# Autodesk Inventor assembly: MeasurementChamber Frame Assembly - Bade v4
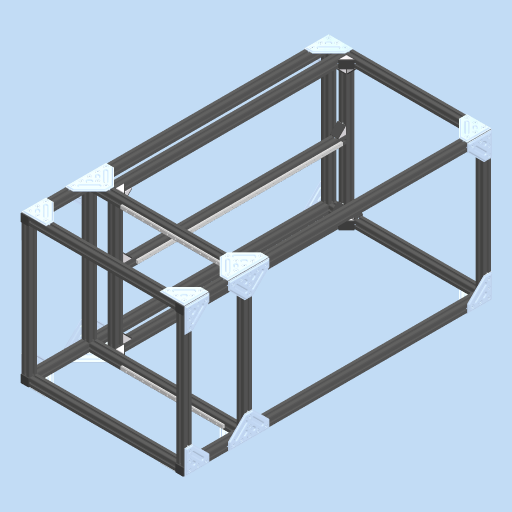
[picture p0: Inventor's stored thumbnail of the model, 512x512]
Saved by Autodesk Inventor 2023.2 (Build 272271000, 271)
## iProperties
Created: 2023-11-22
Part Number: MeasurementChamber Frame Assembly - Bade v4
Document SubType Name: Assembly
Designer: Nils Bade
Author: Nils Bade
## Documents named in this file (16)
- C:\Users\nilsb\Documents\Inventor\Projektarbeit-Bade\ITEM\ITEM Frame Assembly - Bade v1.iam
- ITEM Frame Assembly - Bade v1.iam
- C:\Users\nilsb\Documents\Inventor\Projektarbeit-Bade\ITEM\4040 Profile\ITEM T-SLOT 4040 715mm.ipt
- C:\Users\nilsb\Documents\Inventor\Projektarbeit-Bade\ITEM\4040 Profile\ITEM T-SLOT 4040 1500mm.ipt
- C:\Users\nilsb\Documents\Inventor\Projektarbeit-Bade\ITEM\4040 Profile\ITEM T-SLOT 4040 640mm.ipt
- C:\Users\nilsb\Documents\Inventor\Projektarbeit-Bade\ITEM\4040 Profile\ITEM T-SLOT 4040 1127mm.ipt
- C:\Users\nilsb\Documents\Inventor\Projektarbeit-Bade\ITEM\4040 Profile\ITEM T-SLOT 4040 1087mm.ipt
- C:\Users\nilsb\Documents\Inventor\Projektarbeit-Bade\ITEM\ITEM_41115_Winkelsatz_90er.iam
- C:\Users\nilsb\Documents\Inventor\Projektarbeit-Bade\ITEM\ITEM_0070805_T-Knotenblechsatz 8 40 200x120.ipt
- ITEM_0070805_T-Knotenblechsatz 8 40 200x120.ipt
- C:\Users\nilsb\Documents\Inventor\Projektarbeit-Bade\ITEM\ITEM_0070802_90erKnotenblechsatz 8 40 120x120.ipt
- C:\Users\nilsb\Documents\Inventor\Projektarbeit-Bade\ITEM\ITEM_0070805_T-Knotenblechsatz 8 40 200x120_MIR.ipt
- C:\Users\nilsb\Documents\Inventor\Projektarbeit-Bade\ITEM\ITEM_0070802_90erKnotenblechsatz 8 40 120x120_MIR.ipt
- C:\Users\nilsb\Documents\Inventor\Projektarbeit-Bade\RatRig_modified\MGN15 Linear Rail 1000mm - 4040 Assembly.iam
- C:\Users\nilsb\Documents\Inventor\Projektarbeit-Bade\RatRig_modified\MGN15 Linear Rail 500mm - 4040 Assembly.iam
- C:\Users\nilsb\Documents\Inventor\Projektarbeit-Bade\ITEM\ITEM_Abdeckkappe-40x40-schw_2601.ipt
## Components (66 placed, 13 different names)
1. ITEM T-SLOT 4040 1500mm:1 — Passend:162, Passend:163, Fluchtend:165, Passend:165, Fluchtend:19, Fluchtend:20, Passend:174, Fluchtend:166, Fluchtend:195, Passend:192, Passend:225, Passend:226, Passend:227, Passend:228, Passend:232, Passend:233, Passend:234, Passend:246, Passend:247, Passend:249, Passend:250, Passend:265, Fluchtend:267, Fluchtend:268
2. ITEM T-SLOT 4040 1500mm:2 — Passend:166, Passend:167, Passend:168, Fluchtend:167, Fluchtend:171, Passend:183, Passend:185, Fluchtend:188, Fluchtend:228, Passend:223, Passend:229, Passend:230, Fluchtend:233, Passend:238, Fluchtend:235, Passend:240, Passend:242, Passend:257, Fluchtend:259, Passend:262, Fluchtend:261, Fluchtend:262, Passend:263
3. ITEM T-SLOT 4040 1500mm:3 — Fluchtend:168, Passend:176, Passend:178, Passend:181, Fluchtend:193, Passend:190, Fluchtend:196, Fluchtend:200, Passend:266, Fluchtend:265, Fluchtend:266
4. ITEM T-SLOT 4040 1500mm:4 — Passend:177, Fluchtend:169, Passend:179, Fluchtend:170, Passend:184, Fluchtend:186, Fluchtend:187, Fluchtend:189, Passend:186, Fluchtend:197, Fluchtend:198, Passend:191, Fluchtend:201, Passend:193, Symmetrie:1, Fluchtend:238, Passend:256, Fluchtend:263, Fluchtend:264, Passend:264
5. ITEM T-SLOT 4040 715mm:1 — Passend:165, Fluchtend:19, Fluchtend:20, Passend:168, Passend:172, Passend:173, Fluchtend:194, Passend:188, Fluchtend:207, Fluchtend:210, Fluchtend:215, Passend:200, Passend:201, Fluchtend:236, Fluchtend:237
6. ITEM T-SLOT 4040 715mm:2 — Passend:180, Fluchtend:170, Passend:181, Passend:187, Fluchtend:206, Fluchtend:211, Passend:209, Fluchtend:219, Passend:212
7. ITEM T-SLOT 4040 715mm:3 — Fluchtend:171, Passend:182, Passend:183, Passend:231, Passend:236, Passend:237
8. ITEM T-SLOT 4040 715mm:4 — Passend:184, Fluchtend:186, Fluchtend:187
9. ITEM T-SLOT 4040 715mm:5 — Passend:185, Fluchtend:188, Fluchtend:190, Passend:195, Passend:216, Fluchtend:227, Passend:224, Fluchtend:229
10. ITEM T-SLOT 4040 715mm:6 — Fluchtend:189, Passend:186, Fluchtend:190, Passend:189, Fluchtend:199, Fluchtend:202, Passend:222
11. ITEM T-SLOT 4040 640mm:1 — Passend:171, Passend:172, Fluchtend:167, Passend:175, Fluchtend:169, Passend:179, Fluchtend:205, Fluchtend:212, Fluchtend:213, Passend:241, Passend:243
12. ITEM T-SLOT 4040 640mm:2 — Passend:170, Passend:173, Passend:175, Fluchtend:191, Fluchtend:192, Fluchtend:209, Fluchtend:214, Passend:202, Fluchtend:216, Passend:203, Fluchtend:217, Passend:205, Fluchtend:218, Passend:207, Passend:208, Fluchtend:220, Fluchtend:221
13. ITEM T-SLOT 4040 640mm:3 — Passend:169, Passend:174, Fluchtend:166, Passend:178, Passend:248
14. ITEM T-SLOT 4040 640mm:4 — Passend:194, Passend:195, Fluchtend:203, Fluchtend:208, Passend:215, Passend:217, Passend:219, Fluchtend:225
15. ITEM T-SLOT 4040 640mm:5 — Fluchtend:199, Fluchtend:200, Passend:192
16. ITEM T-SLOT 4040 640mm:6 — Fluchtend:201, Passend:193, Fluchtend:202, Fluchtend:231
17. ITEM T-SLOT 4040 640mm:7 — Fluchtend:197, Fluchtend:198, Passend:191, Fluchtend:234, Passend:239
18. ITEM T-SLOT 4040 640mm:8 — Fluchtend:195, Passend:190, Fluchtend:196, Fluchtend:232, Passend:235
19. ITEM T-SLOT 4040 1127mm:2 — Fluchtend:192, Fluchtend:193, Passend:187, Passend:189, Passend:210, Passend:211, Passend:220, Passend:221, Fluchtend:226
20. ITEM T-SLOT 4040 1127mm:1 — Fluchtend:191, Fluchtend:194, Passend:188, Passend:194, Fluchtend:203, Passend:199, Passend:204, Passend:213, Passend:214, Fluchtend:222, Fluchtend:223
21. ITEM T-SLOT 4040 1087mm:1 — Passend:206, Passend:218, Fluchtend:224, Passend:254, Passend:255
22. ITEM_Abdeckkappe-40x40-schw_2601:1 — Fluchtend:261, Fluchtend:262, Passend:263
23. ITEM_Abdeckkappe-40x40-schw_2601:2 — Fluchtend:263, Fluchtend:264, Passend:264
24. ITEM_Abdeckkappe-40x40-schw_2601:3 — Passend:265, Fluchtend:267, Fluchtend:268
25. ITEM_Abdeckkappe-40x40-schw_2601:4 — Passend:266, Fluchtend:265, Fluchtend:266
26. ITEM_41115_Winkelsatz_90er:1 [sub-assembly] — Fluchtend:215, Passend:199, Passend:200
27. ITEM_41115_Winkelsatz_90er:2 [sub-assembly] — Passend:203, Fluchtend:217, Passend:204
28. ITEM_41115_Winkelsatz_90er:3 [sub-assembly] — Passend:201, Passend:202, Fluchtend:216
29. ITEM_41115_Winkelsatz_90er:4 [sub-assembly] — Passend:205, Passend:206, Fluchtend:218
30. ITEM_41115_Winkelsatz_90er:5 [sub-assembly] — Passend:207, Fluchtend:220, Passend:211
31. ITEM_41115_Winkelsatz_90er:6 [sub-assembly] — Passend:208, Fluchtend:221, Passend:212
32. ITEM_41115_Winkelsatz_90er:7 [sub-assembly] — Passend:209, Passend:210, Fluchtend:219
33. ITEM_41115_Winkelsatz_90er:8 [sub-assembly] — Passend:213, Fluchtend:223, Passend:216
34. ITEM_41115_Winkelsatz_90er:9 [sub-assembly] — Passend:214, Passend:215, Fluchtend:222
35. ITEM_41115_Winkelsatz_90er:10 [sub-assembly] — Passend:217, Passend:218, Fluchtend:224
36. ITEM_41115_Winkelsatz_90er:11 [sub-assembly] — Passend:219, Passend:220, Fluchtend:225
37. ITEM_41115_Winkelsatz_90er:12 [sub-assembly] — Passend:221, Passend:222, Fluchtend:226
38. ITEM_0070805_T-Knotenblechsatz 8 40 200x120:1 — Passend:224, Passend:225, Passend:226
39. ITEM_0070805_T-Knotenblechsatz 8 40 200x120:2 — Fluchtend:227, Fluchtend:228, Passend:223
40. ITEM_0070805_T-Knotenblechsatz 8 40 200x120:3 — Fluchtend:229, Passend:227, Passend:228
41. ITEM_0070805_T-Knotenblechsatz 8 40 200x120:4 — Passend:229, Fluchtend:231, Passend:230
42. ITEM_0070802_90erKnotenblechsatz 8 40 120x120:1 — Passend:231, Passend:232, Passend:233
43. ITEM_0070802_90erKnotenblechsatz 8 40 120x120:2 — Passend:234, Fluchtend:232, Passend:235
44. ITEM_0070802_90erKnotenblechsatz 8 40 120x120:3 — Fluchtend:234, Passend:238, Passend:239
45. ITEM_0070802_90erKnotenblechsatz 8 40 120x120:4 — Passend:236, Fluchtend:233, Passend:237
46. ITEM_0070802_90erKnotenblechsatz 8 40 120x120:5 — Fluchtend:235, Fluchtend:236, Passend:240
47. ITEM_0070802_90erKnotenblechsatz 8 40 120x120:6 — Passend:246, Fluchtend:237, Passend:250
48. ITEM_0070802_90erKnotenblechsatz 8 40 120x120:7 — Passend:241, Passend:242, Passend:243
49. ITEM_0070802_90erKnotenblechsatz 8 40 120x120:8 — Passend:247, Passend:248, Passend:249
50. ITEM_0070805_T-Knotenblechsatz 8 40 200x120_MIR:1
51. ITEM_0070805_T-Knotenblechsatz 8 40 200x120_MIR:2
52. ITEM_0070805_T-Knotenblechsatz 8 40 200x120_MIR:3
53. ITEM_0070805_T-Knotenblechsatz 8 40 200x120_MIR:4
54. ITEM_0070802_90erKnotenblechsatz 8 40 120x120_MIR:1
55. ITEM_0070802_90erKnotenblechsatz 8 40 120x120_MIR:2
56. ITEM_0070802_90erKnotenblechsatz 8 40 120x120_MIR:3
57. ITEM_0070802_90erKnotenblechsatz 8 40 120x120_MIR:4
58. ITEM_0070802_90erKnotenblechsatz 8 40 120x120_MIR:5
59. ITEM_0070802_90erKnotenblechsatz 8 40 120x120_MIR:6
60. ITEM_0070802_90erKnotenblechsatz 8 40 120x120_MIR:7
61. ITEM_0070802_90erKnotenblechsatz 8 40 120x120_MIR:8
62. MGN15 Linear Rail 1000mm - 4040 Assembly:1 [sub-assembly] — Passend:253, Fluchtend:238, Passend:256
63. MGN15 Linear Rail 1000mm - 4040 Assembly:2 [sub-assembly] — Passend:252, Passend:257, Fluchtend:259
64. MGN15 Linear Rail 1000mm - 4040 Assembly:3 [sub-assembly] — Passend:251, Passend:254, Passend:255
65. MGN15 Linear Rail 500mm - 4040 Assembly:1 [sub-assembly] — Passend:262
66. MGN15 Linear Rail 500mm - 4040 Assembly:2 [sub-assembly]
## Relationships (180: Mate 105, Flush 74, Symmetry 1)
- Fluchtend:17 [Flush] (1057 mm)
- Passend:156 [Mate]
- Passend:157 [Mate]
- Passend:158 [Mate]
- Passend:159 [Mate]
- Passend:160 [Mate]
- Passend:161 [Mate]
- Passend:162 [Mate]: ITEM T-SLOT 4040 1500mm:1
- Passend:163 [Mate]: ITEM T-SLOT 4040 1500mm:1
- Fluchtend:165 [Flush]: ITEM T-SLOT 4040 1500mm:1
- Passend:165 [Mate]: ITEM T-SLOT 4040 1500mm:1 ↔ ITEM T-SLOT 4040 715mm:1
- Fluchtend:19 [Flush]: ITEM T-SLOT 4040 1500mm:1 ↔ ITEM T-SLOT 4040 715mm:1
- Fluchtend:20 [Flush]: ITEM T-SLOT 4040 1500mm:1 ↔ ITEM T-SLOT 4040 715mm:1
- Passend:166 [Mate]: ITEM T-SLOT 4040 1500mm:2
- Passend:167 [Mate]: ITEM T-SLOT 4040 1500mm:2
- Passend:168 [Mate]: ITEM T-SLOT 4040 1500mm:2 ↔ ITEM T-SLOT 4040 715mm:1
- Passend:169 [Mate]: ITEM T-SLOT 4040 640mm:3
- Passend:170 [Mate]: ITEM T-SLOT 4040 640mm:2
- Passend:171 [Mate]: ITEM T-SLOT 4040 640mm:1
- Passend:172 [Mate]: ITEM T-SLOT 4040 715mm:1 ↔ ITEM T-SLOT 4040 640mm:1
- Passend:173 [Mate]: ITEM T-SLOT 4040 715mm:1 ↔ ITEM T-SLOT 4040 640mm:2
- Passend:174 [Mate]: ITEM T-SLOT 4040 1500mm:1 ↔ ITEM T-SLOT 4040 640mm:3
- Fluchtend:166 [Flush]: ITEM T-SLOT 4040 1500mm:1 ↔ ITEM T-SLOT 4040 640mm:3
- Fluchtend:167 [Flush]: ITEM T-SLOT 4040 1500mm:2 ↔ ITEM T-SLOT 4040 640mm:1
- Passend:175 [Mate] (628 mm): ITEM T-SLOT 4040 640mm:1 ↔ ITEM T-SLOT 4040 640mm:2
- Fluchtend:168 [Flush]: ITEM T-SLOT 4040 1500mm:3
- Passend:176 [Mate]: ITEM T-SLOT 4040 1500mm:3
- Passend:177 [Mate]: ITEM T-SLOT 4040 1500mm:4
- Passend:178 [Mate]: ITEM T-SLOT 4040 1500mm:3 ↔ ITEM T-SLOT 4040 640mm:3
- Fluchtend:169 [Flush]: ITEM T-SLOT 4040 1500mm:4 ↔ ITEM T-SLOT 4040 640mm:1
- Passend:179 [Mate]: ITEM T-SLOT 4040 1500mm:4 ↔ ITEM T-SLOT 4040 640mm:1
- Passend:180 [Mate]: ITEM T-SLOT 4040 715mm:2
- Fluchtend:170 [Flush]: ITEM T-SLOT 4040 1500mm:4 ↔ ITEM T-SLOT 4040 715mm:2
- Passend:181 [Mate]: ITEM T-SLOT 4040 1500mm:3 ↔ ITEM T-SLOT 4040 715mm:2
- Fluchtend:171 [Flush]: ITEM T-SLOT 4040 1500mm:2 ↔ ITEM T-SLOT 4040 715mm:3
- Passend:182 [Mate]: ITEM T-SLOT 4040 715mm:3
- Passend:183 [Mate]: ITEM T-SLOT 4040 1500mm:2 ↔ ITEM T-SLOT 4040 715mm:3
- Passend:184 [Mate]: ITEM T-SLOT 4040 1500mm:4 ↔ ITEM T-SLOT 4040 715mm:4
- Fluchtend:186 [Flush]: ITEM T-SLOT 4040 1500mm:4 ↔ ITEM T-SLOT 4040 715mm:4
- Fluchtend:187 [Flush]: ITEM T-SLOT 4040 1500mm:4 ↔ ITEM T-SLOT 4040 715mm:4
- Passend:185 [Mate]: ITEM T-SLOT 4040 1500mm:2 ↔ ITEM T-SLOT 4040 715mm:5
- Fluchtend:188 [Flush]: ITEM T-SLOT 4040 1500mm:2 ↔ ITEM T-SLOT 4040 715mm:5
- Fluchtend:189 [Flush]: ITEM T-SLOT 4040 1500mm:4 ↔ ITEM T-SLOT 4040 715mm:6
- Passend:186 [Mate]: ITEM T-SLOT 4040 1500mm:4 ↔ ITEM T-SLOT 4040 715mm:6
- Fluchtend:190 [Flush]: ITEM T-SLOT 4040 715mm:5 ↔ ITEM T-SLOT 4040 715mm:6
- Fluchtend:191 [Flush]: ITEM T-SLOT 4040 640mm:2 ↔ ITEM T-SLOT 4040 1127mm:1
- Fluchtend:192 [Flush]: ITEM T-SLOT 4040 640mm:2 ↔ ITEM T-SLOT 4040 1127mm:2
- Fluchtend:193 [Flush]: ITEM T-SLOT 4040 1500mm:3 ↔ ITEM T-SLOT 4040 1127mm:2
- Passend:187 [Mate]: ITEM T-SLOT 4040 715mm:2 ↔ ITEM T-SLOT 4040 1127mm:2
- Fluchtend:194 [Flush]: ITEM T-SLOT 4040 715mm:1 ↔ ITEM T-SLOT 4040 1127mm:1
- Passend:188 [Mate]: ITEM T-SLOT 4040 715mm:1 ↔ ITEM T-SLOT 4040 1127mm:1
- Passend:189 [Mate]: ITEM T-SLOT 4040 715mm:6 ↔ ITEM T-SLOT 4040 1127mm:2
- Fluchtend:195 [Flush]: ITEM T-SLOT 4040 1500mm:1 ↔ ITEM T-SLOT 4040 640mm:8
- Passend:190 [Mate]: ITEM T-SLOT 4040 1500mm:3 ↔ ITEM T-SLOT 4040 640mm:8
- Fluchtend:196 [Flush]: ITEM T-SLOT 4040 1500mm:3 ↔ ITEM T-SLOT 4040 640mm:8
- Fluchtend:197 [Flush]: ITEM T-SLOT 4040 1500mm:4 ↔ ITEM T-SLOT 4040 640mm:7
- Fluchtend:198 [Flush]: ITEM T-SLOT 4040 1500mm:4 ↔ ITEM T-SLOT 4040 640mm:7
- Passend:191 [Mate]: ITEM T-SLOT 4040 1500mm:4 ↔ ITEM T-SLOT 4040 640mm:7
- Fluchtend:199 [Flush]: ITEM T-SLOT 4040 715mm:6 ↔ ITEM T-SLOT 4040 640mm:5
- Fluchtend:200 [Flush]: ITEM T-SLOT 4040 1500mm:3 ↔ ITEM T-SLOT 4040 640mm:5
- Passend:192 [Mate]: ITEM T-SLOT 4040 1500mm:1 ↔ ITEM T-SLOT 4040 640mm:5
- Fluchtend:201 [Flush]: ITEM T-SLOT 4040 1500mm:4 ↔ ITEM T-SLOT 4040 640mm:6
- Passend:193 [Mate]: ITEM T-SLOT 4040 1500mm:4 ↔ ITEM T-SLOT 4040 640mm:6
- Fluchtend:202 [Flush]: ITEM T-SLOT 4040 715mm:6 ↔ ITEM T-SLOT 4040 640mm:6
- Passend:194 [Mate]: ITEM T-SLOT 4040 640mm:4 ↔ ITEM T-SLOT 4040 1127mm:1
- Passend:195 [Mate]: ITEM T-SLOT 4040 715mm:5 ↔ ITEM T-SLOT 4040 640mm:4
- Fluchtend:203 [Flush]: ITEM T-SLOT 4040 640mm:4 ↔ ITEM T-SLOT 4040 1127mm:1
- [Mate]: ITEM T-SLOT 4040 640mm:2 ↔ ITEM T-SLOT 4040 1087mm:1
- [Flush]: ITEM T-SLOT 4040 640mm:2 ↔ ITEM T-SLOT 4040 1087mm:1
- Symmetrie:1: ITEM T-SLOT 4040 1500mm:4
- [Mate]: ITEM T-SLOT 4040 1087mm:1
- Fluchtend:205 [Flush] (21.5 mm): ITEM T-SLOT 4040 640mm:1
- Fluchtend:206 [Flush] (21.5 mm): ITEM T-SLOT 4040 715mm:2
- Fluchtend:207 [Flush] (21.5 mm): ITEM T-SLOT 4040 715mm:1
- Fluchtend:208 [Flush] (35.5 mm): ITEM T-SLOT 4040 640mm:4
- Fluchtend:209 [Flush] (70 mm): ITEM T-SLOT 4040 640mm:2
- Fluchtend:210 [Flush] (51.86 mm): ITEM T-SLOT 4040 715mm:1
- Fluchtend:211 [Flush] (51.86 mm): ITEM T-SLOT 4040 715mm:2
- Fluchtend:212 [Flush] (25.242 mm): ITEM T-SLOT 4040 640mm:1
- Fluchtend:213 [Flush] (47 mm): ITEM T-SLOT 4040 640mm:1
- Fluchtend:214 [Flush] (27 mm): ITEM T-SLOT 4040 640mm:2
- Fluchtend:215 [Flush]: ITEM T-SLOT 4040 715mm:1 ↔ ITEM_41115_Winkelsatz_90er:1
- Passend:199 [Mate]: ITEM T-SLOT 4040 1127mm:1 ↔ ITEM_41115_Winkelsatz_90er:1
- Passend:200 [Mate]: ITEM T-SLOT 4040 715mm:1 ↔ ITEM_41115_Winkelsatz_90er:1
- Passend:201 [Mate]: ITEM T-SLOT 4040 715mm:1 ↔ ITEM_41115_Winkelsatz_90er:3
- Passend:202 [Mate]: ITEM T-SLOT 4040 640mm:2 ↔ ITEM_41115_Winkelsatz_90er:3
- Fluchtend:216 [Flush]: ITEM T-SLOT 4040 640mm:2 ↔ ITEM_41115_Winkelsatz_90er:3
- Passend:203 [Mate]: ITEM T-SLOT 4040 640mm:2 ↔ ITEM_41115_Winkelsatz_90er:2
- Fluchtend:217 [Flush]: ITEM T-SLOT 4040 640mm:2 ↔ ITEM_41115_Winkelsatz_90er:2
- Passend:204 [Mate]: ITEM T-SLOT 4040 1127mm:1 ↔ ITEM_41115_Winkelsatz_90er:2
- Passend:205 [Mate]: ITEM T-SLOT 4040 640mm:2 ↔ ITEM_41115_Winkelsatz_90er:4
- Passend:206 [Mate]: ITEM T-SLOT 4040 1087mm:1 ↔ ITEM_41115_Winkelsatz_90er:4
- Fluchtend:218 [Flush]: ITEM T-SLOT 4040 640mm:2 ↔ ITEM_41115_Winkelsatz_90er:4
- Passend:207 [Mate]: ITEM T-SLOT 4040 640mm:2 ↔ ITEM_41115_Winkelsatz_90er:5
- Passend:208 [Mate]: ITEM T-SLOT 4040 640mm:2 ↔ ITEM_41115_Winkelsatz_90er:6
- Passend:209 [Mate]: ITEM T-SLOT 4040 715mm:2 ↔ ITEM_41115_Winkelsatz_90er:7
- Passend:210 [Mate]: ITEM T-SLOT 4040 1127mm:2 ↔ ITEM_41115_Winkelsatz_90er:7
- Fluchtend:219 [Flush]: ITEM T-SLOT 4040 715mm:2 ↔ ITEM_41115_Winkelsatz_90er:7
- Fluchtend:220 [Flush]: ITEM T-SLOT 4040 640mm:2 ↔ ITEM_41115_Winkelsatz_90er:5
- Fluchtend:221 [Flush]: ITEM T-SLOT 4040 640mm:2 ↔ ITEM_41115_Winkelsatz_90er:6
- Passend:211 [Mate]: ITEM T-SLOT 4040 1127mm:2 ↔ ITEM_41115_Winkelsatz_90er:5
- Passend:212 [Mate]: ITEM T-SLOT 4040 715mm:2 ↔ ITEM_41115_Winkelsatz_90er:6
- Passend:213 [Mate]: ITEM T-SLOT 4040 1127mm:1 ↔ ITEM_41115_Winkelsatz_90er:8
- Passend:214 [Mate]: ITEM T-SLOT 4040 1127mm:1 ↔ ITEM_41115_Winkelsatz_90er:9
- Passend:215 [Mate]: ITEM T-SLOT 4040 640mm:4 ↔ ITEM_41115_Winkelsatz_90er:9
- Fluchtend:222 [Flush]: ITEM T-SLOT 4040 1127mm:1 ↔ ITEM_41115_Winkelsatz_90er:9
- Fluchtend:223 [Flush]: ITEM T-SLOT 4040 1127mm:1 ↔ ITEM_41115_Winkelsatz_90er:8
- Passend:216 [Mate]: ITEM T-SLOT 4040 715mm:5 ↔ ITEM_41115_Winkelsatz_90er:8
- Passend:217 [Mate]: ITEM T-SLOT 4040 640mm:4 ↔ ITEM_41115_Winkelsatz_90er:10
- Passend:218 [Mate]: ITEM T-SLOT 4040 1087mm:1 ↔ ITEM_41115_Winkelsatz_90er:10
- Fluchtend:224 [Flush]: ITEM T-SLOT 4040 1087mm:1 ↔ ITEM_41115_Winkelsatz_90er:10
- Passend:219 [Mate]: ITEM T-SLOT 4040 640mm:4 ↔ ITEM_41115_Winkelsatz_90er:11
- Passend:220 [Mate]: ITEM T-SLOT 4040 1127mm:2 ↔ ITEM_41115_Winkelsatz_90er:11
- Fluchtend:225 [Flush]: ITEM T-SLOT 4040 640mm:4 ↔ ITEM_41115_Winkelsatz_90er:11
- Passend:221 [Mate]: ITEM T-SLOT 4040 1127mm:2 ↔ ITEM_41115_Winkelsatz_90er:12
- Passend:222 [Mate]: ITEM T-SLOT 4040 715mm:6 ↔ ITEM_41115_Winkelsatz_90er:12
- Fluchtend:226 [Flush]: ITEM T-SLOT 4040 1127mm:2 ↔ ITEM_41115_Winkelsatz_90er:12
- Fluchtend:227 [Flush]: ITEM T-SLOT 4040 715mm:5 ↔ ITEM_0070805_T-Knotenblechsatz 8 40 200x120:2
- Fluchtend:228 [Flush]: ITEM T-SLOT 4040 1500mm:2 ↔ ITEM_0070805_T-Knotenblechsatz 8 40 200x120:2
- Passend:223 [Mate]: ITEM T-SLOT 4040 1500mm:2 ↔ ITEM_0070805_T-Knotenblechsatz 8 40 200x120:2
- Passend:224 [Mate]: ITEM T-SLOT 4040 715mm:5 ↔ ITEM_0070805_T-Knotenblechsatz 8 40 200x120:1
- Passend:225 [Mate]: ITEM T-SLOT 4040 1500mm:1 ↔ ITEM_0070805_T-Knotenblechsatz 8 40 200x120:1
- Passend:226 [Mate]: ITEM T-SLOT 4040 1500mm:1 ↔ ITEM_0070805_T-Knotenblechsatz 8 40 200x120:1
- Fluchtend:229 [Flush]: ITEM T-SLOT 4040 715mm:5 ↔ ITEM_0070805_T-Knotenblechsatz 8 40 200x120:3
- Passend:227 [Mate]: ITEM T-SLOT 4040 1500mm:1 ↔ ITEM_0070805_T-Knotenblechsatz 8 40 200x120:3
- Passend:228 [Mate]: ITEM T-SLOT 4040 1500mm:1 ↔ ITEM_0070805_T-Knotenblechsatz 8 40 200x120:3
- Passend:229 [Mate]: ITEM T-SLOT 4040 1500mm:2 ↔ ITEM_0070805_T-Knotenblechsatz 8 40 200x120:4
- Fluchtend:231 [Flush]: ITEM T-SLOT 4040 640mm:6 ↔ ITEM_0070805_T-Knotenblechsatz 8 40 200x120:4
- Passend:230 [Mate]: ITEM T-SLOT 4040 1500mm:2 ↔ ITEM_0070805_T-Knotenblechsatz 8 40 200x120:4
- Passend:231 [Mate]: ITEM T-SLOT 4040 715mm:3 ↔ ITEM_0070802_90erKnotenblechsatz 8 40 120x120:1
- Passend:232 [Mate]: ITEM T-SLOT 4040 1500mm:1 ↔ ITEM_0070802_90erKnotenblechsatz 8 40 120x120:1
- Passend:233 [Mate]: ITEM T-SLOT 4040 1500mm:1 ↔ ITEM_0070802_90erKnotenblechsatz 8 40 120x120:1
- Passend:234 [Mate]: ITEM T-SLOT 4040 1500mm:1 ↔ ITEM_0070802_90erKnotenblechsatz 8 40 120x120:2
- Fluchtend:232 [Flush]: ITEM T-SLOT 4040 640mm:8 ↔ ITEM_0070802_90erKnotenblechsatz 8 40 120x120:2
- Passend:235 [Mate]: ITEM T-SLOT 4040 640mm:8 ↔ ITEM_0070802_90erKnotenblechsatz 8 40 120x120:2
- Passend:236 [Mate]: ITEM T-SLOT 4040 715mm:3 ↔ ITEM_0070802_90erKnotenblechsatz 8 40 120x120:4
- Fluchtend:233 [Flush]: ITEM T-SLOT 4040 1500mm:2 ↔ ITEM_0070802_90erKnotenblechsatz 8 40 120x120:4
- Passend:237 [Mate]: ITEM T-SLOT 4040 715mm:3 ↔ ITEM_0070802_90erKnotenblechsatz 8 40 120x120:4
- Fluchtend:234 [Flush]: ITEM T-SLOT 4040 640mm:7 ↔ ITEM_0070802_90erKnotenblechsatz 8 40 120x120:3
- Passend:238 [Mate]: ITEM T-SLOT 4040 1500mm:2 ↔ ITEM_0070802_90erKnotenblechsatz 8 40 120x120:3
- Passend:239 [Mate]: ITEM T-SLOT 4040 640mm:7 ↔ ITEM_0070802_90erKnotenblechsatz 8 40 120x120:3
- Fluchtend:235 [Flush]: ITEM T-SLOT 4040 1500mm:2 ↔ ITEM_0070802_90erKnotenblechsatz 8 40 120x120:5
- Fluchtend:236 [Flush]: ITEM T-SLOT 4040 715mm:1 ↔ ITEM_0070802_90erKnotenblechsatz 8 40 120x120:5
- Passend:240 [Mate]: ITEM T-SLOT 4040 1500mm:2 ↔ ITEM_0070802_90erKnotenblechsatz 8 40 120x120:5
- Passend:241 [Mate]: ITEM T-SLOT 4040 640mm:1 ↔ ITEM_0070802_90erKnotenblechsatz 8 40 120x120:7
- Passend:242 [Mate]: ITEM T-SLOT 4040 1500mm:2 ↔ ITEM_0070802_90erKnotenblechsatz 8 40 120x120:7
- Passend:243 [Mate]: ITEM T-SLOT 4040 640mm:1 ↔ ITEM_0070802_90erKnotenblechsatz 8 40 120x120:7
- Passend:246 [Mate]: ITEM T-SLOT 4040 1500mm:1 ↔ ITEM_0070802_90erKnotenblechsatz 8 40 120x120:6
- Fluchtend:237 [Flush]: ITEM T-SLOT 4040 715mm:1 ↔ ITEM_0070802_90erKnotenblechsatz 8 40 120x120:6
- Passend:247 [Mate]: ITEM T-SLOT 4040 1500mm:1 ↔ ITEM_0070802_90erKnotenblechsatz 8 40 120x120:8
- Passend:248 [Mate]: ITEM T-SLOT 4040 640mm:3 ↔ ITEM_0070802_90erKnotenblechsatz 8 40 120x120:8
- Passend:249 [Mate]: ITEM T-SLOT 4040 1500mm:1 ↔ ITEM_0070802_90erKnotenblechsatz 8 40 120x120:8
- Passend:250 [Mate]: ITEM T-SLOT 4040 1500mm:1 ↔ ITEM_0070802_90erKnotenblechsatz 8 40 120x120:6
- Passend:251 [Mate]: MGN15 Linear Rail 1000mm - 4040 Assembly:3
- Passend:252 [Mate]: MGN15 Linear Rail 1000mm - 4040 Assembly:2
- Passend:253 [Mate]: MGN15 Linear Rail 1000mm - 4040 Assembly:1
- Passend:254 [Mate]: ITEM T-SLOT 4040 1087mm:1 ↔ MGN15 Linear Rail 1000mm - 4040 Assembly:3
- Passend:255 [Mate]: ITEM T-SLOT 4040 1087mm:1 ↔ MGN15 Linear Rail 1000mm - 4040 Assembly:3
- Fluchtend:238 [Flush]: ITEM T-SLOT 4040 1500mm:4 ↔ MGN15 Linear Rail 1000mm - 4040 Assembly:1
- Passend:256 [Mate]: ITEM T-SLOT 4040 1500mm:4 ↔ MGN15 Linear Rail 1000mm - 4040 Assembly:1
- Passend:257 [Mate]: ITEM T-SLOT 4040 1500mm:2 ↔ MGN15 Linear Rail 1000mm - 4040 Assembly:2
- Fluchtend:259 [Flush]: ITEM T-SLOT 4040 1500mm:2 ↔ MGN15 Linear Rail 1000mm - 4040 Assembly:2
- [Flush]: ITEM T-SLOT 4040 715mm:5 ↔ MGN15 Linear Rail 500mm - 4040 Assembly:1
- [Mate]: ITEM T-SLOT 4040 715mm:5 ↔ MGN15 Linear Rail 500mm - 4040 Assembly:1
- [Flush]: ITEM T-SLOT 4040 715mm:6 ↔ MGN15 Linear Rail 500mm - 4040 Assembly:2
- [Mate]: ITEM T-SLOT 4040 715mm:6 ↔ MGN15 Linear Rail 500mm - 4040 Assembly:2
- [Flush]: MGN15 Linear Rail 500mm - 4040 Assembly:1 ↔ MGN15 Linear Rail 500mm - 4040 Assembly:2
- Passend:262 [Mate] (55 mm): ITEM T-SLOT 4040 1500mm:2 ↔ MGN15 Linear Rail 500mm - 4040 Assembly:1
- Fluchtend:261 [Flush]: ITEM T-SLOT 4040 1500mm:2 ↔ ITEM_Abdeckkappe-40x40-schw_2601:1
- Fluchtend:262 [Flush]: ITEM T-SLOT 4040 1500mm:2 ↔ ITEM_Abdeckkappe-40x40-schw_2601:1
- Passend:263 [Mate]: ITEM T-SLOT 4040 1500mm:2 ↔ ITEM_Abdeckkappe-40x40-schw_2601:1
- Fluchtend:263 [Flush]: ITEM T-SLOT 4040 1500mm:4 ↔ ITEM_Abdeckkappe-40x40-schw_2601:2
- Fluchtend:264 [Flush]: ITEM T-SLOT 4040 1500mm:4 ↔ ITEM_Abdeckkappe-40x40-schw_2601:2
- Passend:264 [Mate]: ITEM T-SLOT 4040 1500mm:4 ↔ ITEM_Abdeckkappe-40x40-schw_2601:2
- Passend:265 [Mate]: ITEM T-SLOT 4040 1500mm:1 ↔ ITEM_Abdeckkappe-40x40-schw_2601:3
- Passend:266 [Mate]: ITEM T-SLOT 4040 1500mm:3 ↔ ITEM_Abdeckkappe-40x40-schw_2601:4
- Fluchtend:265 [Flush]: ITEM T-SLOT 4040 1500mm:3 ↔ ITEM_Abdeckkappe-40x40-schw_2601:4
- Fluchtend:266 [Flush]: ITEM T-SLOT 4040 1500mm:3 ↔ ITEM_Abdeckkappe-40x40-schw_2601:4
- Fluchtend:267 [Flush]: ITEM T-SLOT 4040 1500mm:1 ↔ ITEM_Abdeckkappe-40x40-schw_2601:3
- Fluchtend:268 [Flush]: ITEM T-SLOT 4040 1500mm:1 ↔ ITEM_Abdeckkappe-40x40-schw_2601:3
